# Autodesk Inventor assembly: TelescopeAssembly
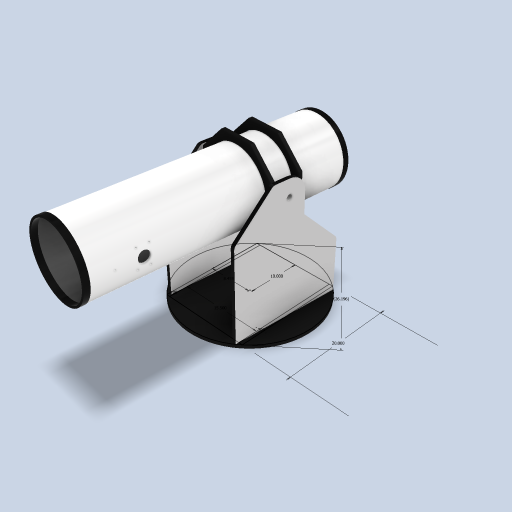
[picture p0: Inventor's stored thumbnail of the model, 512x512]
Saved by Autodesk Inventor 2023 (Build 270158000, 158)
## iProperties
Created: 2022-10-12
Part Number: TelescopeAssembly
Document SubType Name: Assembly
Designer: Nathan
Author: Nathan
## Documents named in this file (6)
- C:\Users\Nathan\Desktop\Senior Project\Schematics\Parts\TelescopeAssembly.iam
- C:\Users\Nathan\Desktop\Senior Project\Schematics\Parts\tube.ipt
- C:\Users\Nathan\Desktop\Senior Project\Schematics\Parts\tubecap.ipt
- C:\Users\Nathan\Desktop\Senior Project\Schematics\Parts\Bracket.ipt
- C:\Users\Nathan\Desktop\Senior Project\Schematics\Parts\base side.ipt
- C:\Users\Nathan\Desktop\Senior Project\Schematics\Parts\base turntable.ipt
## Components (8 placed, 5 different names)
1. tube:1 — Mate:1, Mate:2, Mate:3, Mate:4
2. Telescope Cap:1 — Mate:2, Mate:5, Mate:6
3. Telescope Cap:2 — Mate:1
4. Bracket:1 — Mate:4, Mate:6
5. Bracket:2 — Mate:3, Mate:5, Mate:7, Mate:8
6. base side:1 — Mate:7, Mate:9, Flush:1, Tangent:1, Tangent:2
7. base side:2 — Mate:8, Mate:10, Flush:1
8. base turntable:1 — Mate:9, Mate:10, Tangent:1, Tangent:2
## Relationships (13: Mate 10, Tangent 2, Flush 1)
- Mate:1: tube:1 ↔ Telescope Cap:2
- Mate:2: tube:1 ↔ Telescope Cap:1
- Mate:3: tube:1 ↔ Bracket:2
- Mate:4: tube:1 ↔ Bracket:1
- Mate:5 (-762 mm): Telescope Cap:1 ↔ Bracket:2
- Mate:6 (-889 mm): Telescope Cap:1 ↔ Bracket:1
- Mate:7: Bracket:2 ↔ base side:1
- Mate:8: Bracket:2 ↔ base side:2
- Mate:9: base side:1 ↔ base turntable:1
- Mate:10: base side:2 ↔ base turntable:1
- Flush:1: base side:1 ↔ base side:2
- Tangent:1: base side:1 ↔ base turntable:1
- Tangent:2: base side:1 ↔ base turntable:1
